# Autodesk Inventor assembly: entero
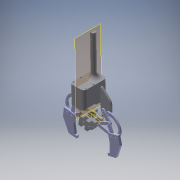
[picture p0: Inventor's stored thumbnail of the model, 180x180]
Saved by Autodesk Inventor 2018 (Build 220112000, 112)
## iProperties
Created: 2018-05-25
Part Number: entero
Document SubType Name: Assembly
Designer: vigus
Author: vigus
## Documents named in this file (7)
- C:\Users\vigus\Documents\gihug\hecatonquiros\cad_models\accesories\gripper\entero.iam
- C:\Users\vigus\Documents\gihug\hecatonquiros\cad_models\tools\gripper\serial_model_0dof\core_attachment.ipt
- C:\Users\vigus\Documents\gihug\hecatonquiros\cad_models\accesories\gripper\Imported Components\garra\garra.ipt
- C:\Users\vigus\Documents\gihug\hecatonquiros\cad_models\accesories\gripper\Imported Components\garra_pilar\garra_pilar.ipt
- C:\Users\vigus\Documents\gihug\hecatonquiros\cad_models\accesories\gripper\Imported Components\garra_pilar_3\garra_pilar_3.ipt
- C:\Users\vigus\Documents\gihug\hecatonquiros\cad_models\tools\gripper\serial_model_0dof\ScrewActuatorGripperCenter.ipt
- C:\Users\vigus\Documents\gihug\hecatonquiros\cad_models\accesories\gripper\triangulobarra_trian.ipt
## Components (10 placed, 6 different names)
1. core_attachment:1 — Mate:2, Mate:3, Mate:6, Mate:7, Mate:13, Mate:14, Mate:15, Mate:16
2. garra:1 — Mate:8, Mate:9, Mate:24
3. garra_pilar:1 — Mate:2, Mate:3, Mate:22, Mate:23
4. garra_pilar_3:1 — Mate:6, Mate:7, Mate:8, Mate:9
5. ScrewActuatorGripperCenter:1 — Mate:28, Mate:29, Mate:30, Mate:31
6. garra:2 — Mate:20, Mate:21, Mate:27
7. garra_pilar:2 — Mate:13, Mate:14, Mate:25, Mate:26
8. garra_pilar_3:2 — Mate:15, Mate:16, Mate:20, Mate:21
9. triangulobarra_trian:1 — Mate:25, Mate:26, Mate:27, Mate:28, Mate:31
10. triangulobarra_trian:2 — Mate:22, Mate:23, Mate:24, Mate:29, Mate:30
## Relationships (22: Mate 22)
- Mate:2: core_attachment:1 ↔ garra_pilar:1
- Mate:3: core_attachment:1 ↔ garra_pilar:1
- Mate:6: core_attachment:1 ↔ garra_pilar_3:1
- Mate:7: core_attachment:1 ↔ garra_pilar_3:1
- Mate:8: garra:1 ↔ garra_pilar_3:1
- Mate:9: garra:1 ↔ garra_pilar_3:1
- Mate:13: core_attachment:1 ↔ garra_pilar:2
- Mate:14: core_attachment:1 ↔ garra_pilar:2
- Mate:15: core_attachment:1 ↔ garra_pilar_3:2
- Mate:16: core_attachment:1 ↔ garra_pilar_3:2
- Mate:20: garra:2 ↔ garra_pilar_3:2
- Mate:21: garra:2 ↔ garra_pilar_3:2
- Mate:22: garra_pilar:1 ↔ triangulobarra_trian:2
- Mate:23: garra_pilar:1 ↔ triangulobarra_trian:2
- Mate:24: garra:1 ↔ triangulobarra_trian:2
- Mate:25: garra_pilar:2 ↔ triangulobarra_trian:1
- Mate:26: garra_pilar:2 ↔ triangulobarra_trian:1
- Mate:27: garra:2 ↔ triangulobarra_trian:1
- Mate:28: ScrewActuatorGripperCenter:1 ↔ triangulobarra_trian:1
- Mate:29: ScrewActuatorGripperCenter:1 ↔ triangulobarra_trian:2
- Mate:30: ScrewActuatorGripperCenter:1 ↔ triangulobarra_trian:2
- Mate:31: ScrewActuatorGripperCenter:1 ↔ triangulobarra_trian:1
